# Autodesk Inventor assembly: talon plate subassy short
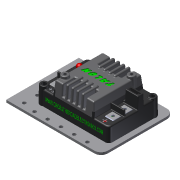
[picture p0: Inventor's stored thumbnail of the model, 180x180]
Saved by Autodesk Inventor 2015 (Build 190159000, 159)
## iProperties
Created: 2015-02-10
Part Number: talon plate subassy short
Document SubType Name: Assembly
Designer: sspriggs
Mass: 55.3223 g
Surface Area: 522.356 cm^2
Volume: 55.3223 cm^3
Density: 1 g/cm^3
Author: sspriggs
## Documents named in this file (3)
- H:\2015\Workspaces\Workspace\electronics parts\talon plate subassy short.iam
- H:\2015\Workspaces\Workspace\electronics parts\talon plate short.ipt
- H:\2015\Workspaces\Workspace\electronics parts\Talon.ipt
## Components (2 placed, 2 different names)
1. talon plate short:1 — Mate:1, Mate:2, Mate:3
2. Talon:1 — Mate:1, Mate:2, Mate:3
## Relationships (3: Mate 3)
- Mate:1: talon plate short:1 ↔ Talon:1
- Mate:2: talon plate short:1 ↔ Talon:1
- Mate:3: talon plate short:1 ↔ Talon:1
